# Autodesk Inventor assembly: Emblem
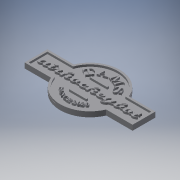
[picture p0: Inventor's stored thumbnail of the model, 180x180]
Saved by Autodesk Inventor 2019.3 (Build 233278000, 278)
## iProperties
Created: 2020-09-20
Part Number: Emblem
Material: Generisch
Document SubType Name: Assembly
Designer: Nicolas Frick
Author: Nicolas Frick
## Documents named in this file (3)
- C:\Users\Nicolas Frick\Sync\OneDrive\airhockeybot\mechanical_design\inventor\Emblem.iam
- C:\Users\Nicolas Frick\Sync\OneDrive\airhockeybot\mechanical_design\inventor\Emblem.ipt
- C:\Users\Nicolas Frick\Sync\OneDrive\airhockeybot\mechanical_design\inventor\Emblem_script.ipt
## Components (2 placed, 2 different names)
1. Emblem:1 — Passend:1, Fluchtend:1, Fluchtend:2, Passend:2, Fluchtend:3, Fluchtend:4
2. Emblem_script:1 — Passend:2, Fluchtend:3, Fluchtend:4
## Relationships (6: Flush 4, Mate 2)
- Passend:1 [Mate]: Emblem:1
- Fluchtend:1 [Flush]: Emblem:1
- Fluchtend:2 [Flush]: Emblem:1
- Passend:2 [Mate]: Emblem:1 ↔ Emblem_script:1
- Fluchtend:3 [Flush]: Emblem:1 ↔ Emblem_script:1
- Fluchtend:4 [Flush]: Emblem:1 ↔ Emblem_script:1
